# Autodesk Inventor assembly: s-assy-cover-left
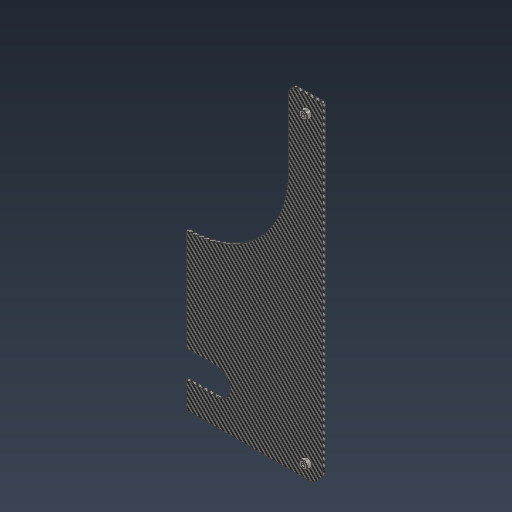
[picture p0: Inventor's stored thumbnail of the model, 512x512]
Saved by Autodesk Inventor 2021 (Build 250183000, 183)
## iProperties
Created: 2021-08-05
Part Number: s-assy-cover-left
Document SubType Name: Assembly
Designer: yuta0
Author: yuta0
## Documents named in this file (4)
- C:\Users\yuta0\Documents\GitHub\catchrobo_hardware\assy-robot\s-assy-cover-left.iam
- C:\Users\yuta0\Documents\GitHub\catchrobo_hardware\assy-robot\carbon_plate5.ipt
- C:\Users\yuta0\Documents\GitHub\catchrobo_hardware\assy-robot\CB3-5.ipt
- C:\Users\yuta0\Documents\GitHub\catchrobo_hardware\assy-robot\LBNR3.ipt
## Components (5 placed, 3 different names)
1. carbon_plate5:1 — メイト:5, メイト:6, メイト:8
2. LBNR3:1 — メイト:7, メイト:8
3. CB3-5:1 — メイト:5, メイト:6, メイト:7
4. LBNR3:2
5. CB3-5:2
## Component patterns: (2 elements, first: LBNR3:1 + CB3-5:1)
## Relationships (4: Mate 4)
- メイト:5 [Mate]: carbon_plate5:1 ↔ CB3-5:1
- メイト:6 [Mate]: carbon_plate5:1 ↔ CB3-5:1
- メイト:7 [Mate]: LBNR3:1 ↔ CB3-5:1
- メイト:8 [Mate]: carbon_plate5:1 ↔ LBNR3:1
